# Autodesk Inventor assembly: Swing Bin Master - SB
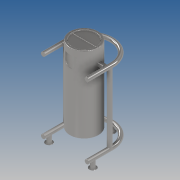
[picture p0: Inventor's stored thumbnail of the model, 180x180]
Saved by Autodesk Inventor 2021.1 (Build 251245000, 245)
## iProperties
Created: 2020-08-18
Part Number: Swing Bin Master - SB
Document SubType Name: Assembly
Designer: CS
Author: CS
## Documents named in this file (11)
- D:\Sam\Inventor\Projects 2021\Inventor Forum\Adaptivity failure\Swing Bin Master - SB.iam
- D:\Sam\Inventor\Projects 2021\Inventor Forum\Adaptivity failure\Bin - SB.ipt
- D:\Sam\Inventor\Projects 2021\Inventor Forum\Adaptivity failure\Upper Frame - SB.ipt
- D:\Sam\Inventor\Projects 2021\Inventor Forum\Adaptivity failure\Vertical Frame - SB.ipt
- D:\Sam\Inventor\Projects 2021\Inventor Forum\Adaptivity failure\Swivel - SB.ipt
- D:\Sam\Inventor\Projects 2021\Inventor Forum\Adaptivity failure\Swivel Cup - SB.ipt
- D:\Sam\Inventor\Projects 2021\Inventor Forum\Adaptivity failure\Tube Cap - SB.ipt
- D:\Sam\Inventor\Projects 2021\Inventor Forum\Adaptivity failure\Bin Lid - SB.ipt
- D:\Sam\Inventor\Projects 2021\Inventor Forum\Adaptivity failure\Front Leg - SB.ipt
- D:\Sam\Inventor\Projects 2021\Inventor Forum\Adaptivity failure\Back Leg - SB.ipt
- D:\Sam\Inventor\Projects 2021\Inventor Forum\Adaptivity failure\Foot - SB.ipt
## Components (20 placed, 10 different names)
1. Bin - SB:1 — Flush:4, Flush:5, Flush:6, Flush:7, Mate:2, Flush:8, Flush:10, Tangent:1, Angle:1, Angle:2
2. Upper Frame - SB:1 — Insert:1, Mate:7
3. Vertical Frame - SB:1 — Mate:1, Symmetry:1
4. Vertical Frame - SB:2 — Symmetry:1, Flush:3
5. Upper Frame - SB:2 — Flush:1, Flush:2, Mate:1, Insert:2, Insert:3
6. Swivel - SB:1 — Flush:5, Flush:6, Flush:7, Symmetry:2, Mate:6, Mate:7
7. Swivel - SB:2 — Symmetry:2, Mate:2, Flush:8
8. Swivel Cup - SB:1
9. Swivel Cup - SB:2 — Mate:3, Mate:4, Flush:9
10. Tube Cap - SB:1
11. Tube Cap - SB:2 — Insert:1
12. Tube Cap - SB:3 — Insert:2
13. Tube Cap - SB:4 — Insert:3
14. Bin Lid - SB:1 — Flush:10, Mate:5, Tangent:1, Angle:2
15. Front Leg - SB:1 — Symmetry:3
16. Front Leg - SB:2 — Flush:11, Mate:8, Symmetry:3, Insert:5
17. Back Leg - SB:1 — Insert:4
18. Foot - SB:1
19. Foot - SB:2 — Insert:4
20. Foot - SB:3 — Insert:5
## Relationships (30: Flush 11, Mate 8, Insert 5, Symmetry 3, Angle 2, Tangent 1)
- Flush:1: Upper Frame - SB:2
- Flush:2: Upper Frame - SB:2
- Mate:1: Vertical Frame - SB:1 ↔ Upper Frame - SB:2
- Symmetry:1: Vertical Frame - SB:1 ↔ Vertical Frame - SB:2
- Flush:3: Vertical Frame - SB:2
- Flush:4: Bin - SB:1
- Flush:5: Bin - SB:1 ↔ Swivel - SB:1
- Flush:6: Bin - SB:1 ↔ Swivel - SB:1
- Flush:7: Bin - SB:1 ↔ Swivel - SB:1
- Symmetry:2: Swivel - SB:1 ↔ Swivel - SB:2
- Mate:2: Bin - SB:1 ↔ Swivel - SB:2
- Flush:8: Bin - SB:1 ↔ Swivel - SB:2
- Mate:3: Swivel Cup - SB:2
- Mate:4: Swivel Cup - SB:2
- Flush:9: Swivel Cup - SB:2
- Insert:1: Upper Frame - SB:1 ↔ Tube Cap - SB:2
- Insert:2: Upper Frame - SB:2 ↔ Tube Cap - SB:3
- Insert:3: Upper Frame - SB:2 ↔ Tube Cap - SB:4
- Flush:10: Bin - SB:1 ↔ Bin Lid - SB:1
- Mate:5: Bin Lid - SB:1
- Tangent:1: Bin - SB:1 ↔ Bin Lid - SB:1
- Mate:6: Swivel - SB:1
- Mate:7: Upper Frame - SB:1 ↔ Swivel - SB:1
- Angle:1 (0 deg): Bin - SB:1
- Angle:2 (0 deg): Bin - SB:1 ↔ Bin Lid - SB:1
- Flush:11: Front Leg - SB:2
- Mate:8: Front Leg - SB:2
- Symmetry:3: Front Leg - SB:1 ↔ Front Leg - SB:2
- Insert:4: Back Leg - SB:1 ↔ Foot - SB:2
- Insert:5: Front Leg - SB:2 ↔ Foot - SB:3
